# Autodesk Inventor assembly: SpecSUPERGEAR2
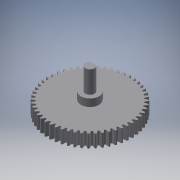
[picture p0: Inventor's stored thumbnail of the model, 180x180]
Saved by Autodesk Inventor 2016 (Build 200138000, 138)
## iProperties
Created: 2018-03-03
Part Number: SpecSUPERGEAR2
Document SubType Name: Assembly
Designer: Simon
Author: Simon
## Documents named in this file (3)
- D:\Cad\Gymnasieprojekt\SpecSUPERGEAR2.iam
- D:\Cad\Gymnasieprojekt\SUPERGEAR2.ipt
- D:\Cad\Gymnasieprojekt\KruggHolder2.ipt
## Components (2 placed, 2 different names)
1. SUPERGEAR2:1 — Insert:1
2. KruggHolder2:1 — Insert:1
## Relationships (1: Insert 1)
- Insert:1: SUPERGEAR2:1 ↔ KruggHolder2:1
